# Autodesk Inventor assembly: MSK01-06A
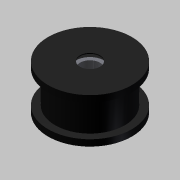
[picture p0: Inventor's stored thumbnail of the model, 180x180]
Saved by Autodesk Inventor 2013 (Build 170138000, 138)
## iProperties
Created: 2012-01-24
Part Number: MSK01-06A
Document SubType Name: Assembly
Designer: ERF
Description: Smooth Idler Assembly
Stock Number: B30041_ASSY
Author: ERF
Title: Smooth Idler Assembly
## Documents named in this file (4)
- C:\Users\Brett\Documents\Autodesk\Projects\Shapeoko_v1i\Assemblies\MSK01-06A.iam
- C:\Users\Brett\Documents\Autodesk\Projects\Shapeoko_v1i\Parts\BEARING_5_16_5.ipt
- C:\Users\Brett\Documents\Autodesk\Projects\Shapeoko_v1i\Parts\B18026.ipt
- C:\Users\Brett\Documents\Autodesk\Projects\Shapeoko_v1i\Parts\B17023.ipt
## Components (4 placed, 3 different names)
1. BEARING_5_16_5:1 — Flush:1, Flush:2
2. BEARING_5_16_5:2 — Insert:1, Mate:1
3. B18026:1 — Flush:1, Insert:1
4. B17023:1 — Mate:1, Flush:2
## Relationships (4: Flush 2, Insert 1, Mate 1)
- Flush:1: BEARING_5_16_5:1 ↔ B18026:1
- Insert:1: BEARING_5_16_5:2 ↔ B18026:1
- Mate:1: BEARING_5_16_5:2 ↔ B17023:1
- Flush:2 (-1.4 mm): BEARING_5_16_5:1 ↔ B17023:1
